# Autodesk Inventor assembly: MX-64T+idle.ipt
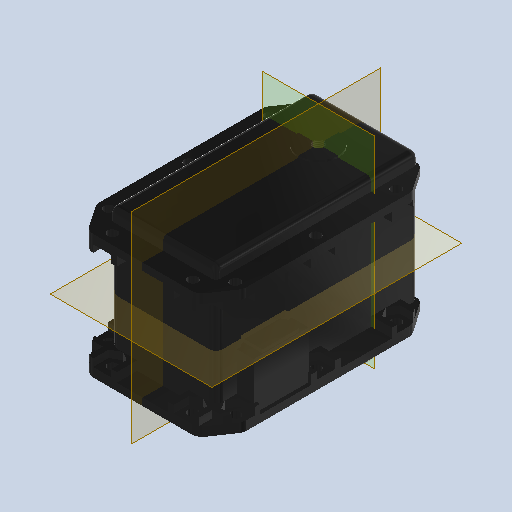
[picture p0: Inventor's stored thumbnail of the model, 512x512]
Saved by Autodesk Inventor 2024.3 (Build 283343000, 343)
## iProperties
Created: 2022-08-09
Part Number: MX-64T+idle.ipt
Document SubType Name: Assembly
Designer: 박지훈
Author: 박지훈
## Documents named in this file (3)
- C:\Users\구지현\Desktop\19th_intern_kdy_fight_robot\부품\ROBOTIS(Inventor 2024 ver.)\다이나믹셀\MX-64T+idle.ipt.iam
- C:\Users\구지현\Desktop\19th_intern_kdy_fight_robot\부품\ROBOTIS(Inventor 2024 ver.)\다이나믹셀\MX-64T.ipt
- C:\Users\구지현\Desktop\19th_intern_kdy_fight_robot\부품\ROBOTIS(Inventor 2024 ver.)\아이들러\64아이들러.iam
## Components (2 placed, 2 different names)
1. MX-64T:1 — 삽입:1
2. 64아이들러:1 [sub-assembly] — 삽입:1
## Relationships (1: Insert 1)
- 삽입:1 [Insert] (0.06 mm): MX-64T:1 ↔ 64아이들러:1
